# Autodesk Inventor assembly: THK-SR15W-1SS520200PB1021B231_5000
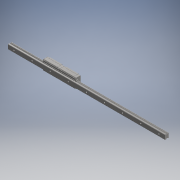
[picture p0: Inventor's stored thumbnail of the model, 180x180]
Saved by Autodesk Inventor 2016 (Build 200138000, 138)
## iProperties
Category: PARTsolutions
Company: THK
Created: 2015-05-03
Part Number: THK-SR15W-1SS520200PB1021B231_5000
Catalog Web Link: www.cadenas.de
Description: Standard Type SR-W/T-
Vendor: THK
Document SubType Name: Assembly
Designer: PARTuser1
Manufacturer: THK
PSOL_IDENT_0: {$CADENAS_DATA\23d-libs\thk\linear_motion_systems\lm_guide\lm_guide\lm_guide_sr\sr_wt_asmtab.prj},24
PSOL_IDENT_1: 3 {VTYP=3D},{STYP=ASSTAB},{NB=SR15W1SS520200PB1021B231.5000},{LINA=SR15 W 1 SS +520L},{NN=Standard T
PSOL_IDENT_2: ype SR-W/T},{DATE=10.03.2011 08:12:40},{GEOMDATE=10.03.2009},{VERSION=},{LINEID=10},{LINESUBID=-1},{
PSOL_IDENT_3: WBVAR=NOB,SO,L,G,GX,NR,POR,GPJ,P1,P2,P3,P4}  {NB=SR15W1SS520200PB1021B231.5000},{LINA=SR15 W 1 SS +5
PSOL_IDENT_4: 20L},{KT=DUMMY},{MN=SR15W},{PD=160},{NOB=1},{SO=SS},{L=520.0},{G=},{INFO=InfoText},{SO1='SS','SS- Wi
PSOL_IDENT_5: th end, side seals','UU','UU- With end seals (on both ends)','DD','DD- With double, side, inner seal
PSOL_IDENT_6: s','ZZ','ZZ- With end, side, inner seals and metal scrapers','KK','KK- With double, side, inner seal
PSOL_IDENT_7: s and metal scrapers'},{LX=57},{EX=5},{LLL=62},{L0=62},{LMIN=63},{LMINX=63},{GG='', 'Symmetrical (G1=
PSOL_IDENT_8: G2)', 'A', 'Asymmetrical'},{GX=20},{GX2=20},{GX1=20},{RC1=No connection},{NR=},{POR=0},{POR1=0,[0:0]
PSOL_IDENT_9: },{GPJ=PB1021B},{INFO1=InfoText},{P1=231.5},{P2=0},{P3=0},{P4=0},{LEND=7200},{LPORM=44.00},{LPORX=10
PSOL_IDENT_10: 00.00},{GPJ1=<'PB1021B', 'PB1021B'>, '', 'None'},{PSM1=0},{PSM2=0},{PSM3=0},{PSM4=0},{PS1=463},{PS2=
PSOL_IDENT_11: 0},{PS3=0},{PS4=0},{PSX2=0},{PSX3=0},{PSX4=0},{LTR=57.00},{L1=39.50},{F=60.00},{D1=3.50},{D2=6.00},{
PSOL_IDENT_12: HM=4.50},{MAXL=2500.00},{GMIN=4},{GMX=20},{GMAX1=8.533333},{G1=12},{G2=12},{NX=1},{LT=2400.00},{A=9}
PSOL_IDENT_13: ,{LF=522},{LM=520},{LL=518},{AA=8.166667},{GA=20.00},{GMAX=36},{RCX=},{H3=4.50},{ND=1.000},{ON=SR15
PSOL_IDENT_14: W},{ON1= },{NRR=},{L4=1.5},{PPATH=sr_wt/sr_wt_asmtpl.prj},{INFOX=block1_1_},{INFOX2=dim_},{PD1=231.5
PSOL_IDENT_15: },{LMIN11=160}
SUPPLIER: THK
ARTICLENO: SR15W1SS520200PB1021B231.5000
BOMINFO: SR15 W 1 SS +520L
CREATOR: CADENAS GmbH
Title: SR15 W 1 SS +520L
Author: Cadenas PARTsolutions
## Documents named in this file (3)
- C:\Users\ax\Documents\Inventor\mintplacer\THK-SR15W-1SS520200PB1021B231_5000.iam
- C:\Users\ax\Documents\Inventor\mintplacer\SR15W52020_Track.ipt
- C:\Users\ax\Documents\Inventor\mintplacer\SR15WSSPB1021B_Slide15_150.ipt
## Components (3 placed, 2 different names)
1. SR15W52020_Track:1 — Slider:1
2. SR15WSSPB1021B_Slide15_150:1 — Slider:1, Mate:1
3. SR15WSSPB1021B_Slide15_150:2 — Mate:1
## Relationships (2: TranslationJoint 1, Mate 1)
- Slider:1 [TranslationJoint]: SR15W52020_Track:1 ↔ SR15WSSPB1021B_Slide15_150:1
- Mate:1: SR15WSSPB1021B_Slide15_150:1 ↔ SR15WSSPB1021B_Slide15_150:2
